# Autodesk Inventor assembly: Assembly suelo
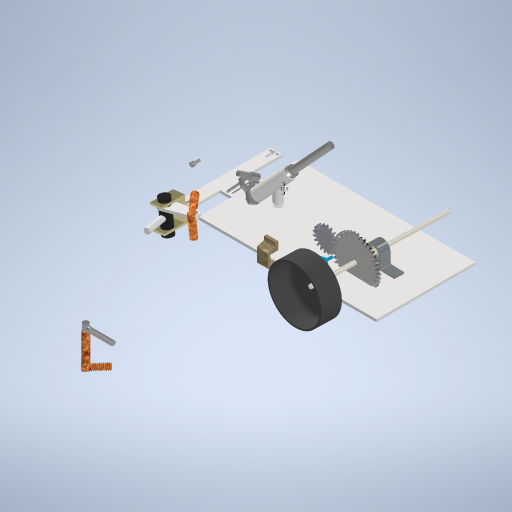
[picture p0: Inventor's stored thumbnail of the model, 512x512]
Saved by Autodesk Inventor 2024 (Build 280153020, 153B)
## iProperties
Created: 2023-05-06
Part Number: Assembly suelo
Document SubType Name: Assembly
Designer: Diego
Author: Diego
## Documents named in this file (20)
- C:\Users\Diego\Videos\Kart_micros\Assembly suelo.iam
- C:\Users\Diego\Videos\Kart_micros\suelo_imp.ipt
- C:\Users\Diego\Videos\Kart_micros\tornillo_5_5_10_5.ipt
- C:\Users\Diego\Videos\Kart_micros\llanta_1.ipt
- C:\Users\Diego\Videos\Kart_micros\tornillo_7_21.ipt
- C:\Users\Diego\Videos\Kart_micros\movil_llanta.ipt
- C:\Users\Diego\Videos\Kart_micros\conex_llantamov.ipt
- C:\Users\Diego\Videos\Kart_micros\soporte1.ipt
- C:\Users\Diego\Videos\Kart_micros\barra_volante.ipt
- C:\Users\Diego\Videos\Kart_micros\union_movllantas.ipt
- C:\Users\Diego\Videos\Kart_micros\Tubo_steering.ipt
- C:\Users\Diego\Videos\Kart_micros\Tubo_steering22.ipt
- C:\Users\Diego\Videos\Kart_micros\Rear_motor.ipt
- C:\Users\Diego\Videos\Kart_micros\Rear_tubo.ipt
- C:\Users\Diego\Videos\Kart_micros\Soporte_cojinete.ipt
- C:\Users\Diego\Videos\Kart_micros\cojinete.ipt
- C:\Users\Diego\Videos\Kart_micros\barra_motores.ipt
- C:\Users\Diego\Videos\Kart_micros\motor.ipt
- C:\Users\Diego\Videos\Kart_micros\soporte_motor.ipt
- C:\Users\Diego\Videos\Kart_micros\ruedas_traseras.ipt
## Components (21 placed, 19 different names)
1. suelo_imp:1 — Rigid:3, Rotational:1, Rotation:1, Rotational:2, Cylindrical:7
2. tornillo_5_5_10_5:1
3. llanta_1:1 — Rotational:1, Cylindrical:1
4. tornillo_7_21:1 — Rigid:3
5. movil_llanta:1 — Cylindrical:1, Rigid:4
6. conex_llantamov:1 — Rigid:4, Cylindrical:8
7. soporte1:1 — Cylindrical:2, Rotation:1, Cylindrical:7
8. barra_volante:1 — Cylindrical:2, Rigid:5
9. union_movllantas:1 — Rigid:5, Cylindrical:9
10. Tubo_steering:1 — Cylindrical:3
11. Tubo_steering22:1 — Cylindrical:3
12. Rear_motor:1
13. Rear_tubo:1 — Cylindrical:6
14. Soporte_cojinete:1 — Rotational:2, Cylindrical:4
15. cojinete:1 — Cylindrical:4, Cylindrical:5
16. barra_motores:1 — Cylindrical:5, Cylindrical:6, Rotational:3
17. motor:1
18. Tubo_steering:2 — Cylindrical:8
19. Tubo_steering22:2 — Cylindrical:9
20. soporte_motor:1
21. ruedas_traseras:1 — Rotational:3
## Relationships (16: CylindricalJoint 9, WeldJoint 3, RevoluteJoint 3, RelateRotation 1)
- Rigid:3 [WeldJoint]: suelo_imp:1 ↔ tornillo_7_21:1
- Rotational:1 [RevoluteJoint]: suelo_imp:1 ↔ llanta_1:1
- Cylindrical:1: llanta_1:1 ↔ movil_llanta:1
- Rigid:4 [WeldJoint] (12 mm): movil_llanta:1 ↔ conex_llantamov:1
- Cylindrical:2: soporte1:1 ↔ barra_volante:1
- Rotation:1 [RelateRotation] (1 ul): suelo_imp:1 ↔ soporte1:1
- Rigid:5 [WeldJoint]: barra_volante:1 ↔ union_movllantas:1
- Cylindrical:3: Tubo_steering:1 ↔ Tubo_steering22:1
- Rotational:2 [RevoluteJoint]: suelo_imp:1 ↔ Soporte_cojinete:1
- Cylindrical:4: Soporte_cojinete:1 ↔ cojinete:1
- Cylindrical:5: cojinete:1 ↔ barra_motores:1
- Cylindrical:6: Rear_tubo:1 ↔ barra_motores:1
- Cylindrical:7: suelo_imp:1 ↔ soporte1:1
- Cylindrical:8: conex_llantamov:1 ↔ Tubo_steering:2
- Cylindrical:9: union_movllantas:1 ↔ Tubo_steering22:2
- Rotational:3 [RevoluteJoint] (6 mm): barra_motores:1 ↔ ruedas_traseras:1
